# Autodesk Inventor assembly: LegAssembly
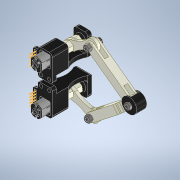
[picture p0: Inventor's stored thumbnail of the model, 180x180]
Saved by Autodesk Inventor 2022 (Build 260153000, 153)
## iProperties
Created: 2021-12-08
Part Number: LegAssembly
Document SubType Name: Assembly
Designer: JK
Author: JK
## Documents named in this file (10)
- C:\Users\JK\Documents\Inventor\N20 Leg Actuator\N20-Leg-Actuator\CADfiles\N20 Leg\LegAssembly.iam
- C:\Users\JK\Documents\Inventor\N20 Leg Actuator\N20-Leg-Actuator\CADfiles\N20Module\N20Module.iam
- C:\Users\JK\Documents\Inventor\N20 Leg Actuator\N20-Leg-Actuator\CADfiles\N20 Leg\ShortLink.ipt
- C:\Users\JK\Documents\Inventor\N20 Leg Actuator\N20-Leg-Actuator\CADfiles\N20 Leg\683zz.ipt
- C:\Users\JK\Documents\Inventor\N20 Leg Actuator\N20-Leg-Actuator\CADfiles\N20 Leg\LinkB.ipt
- C:\Users\JK\Documents\Inventor\N20 Leg Actuator\N20-Leg-Actuator\CADfiles\N20 Leg\LinkA.ipt
- C:\Users\JK\Documents\Inventor\N20 Leg Actuator\N20-Leg-Actuator\CADfiles\N20Module\N20Module_MIR.iam
- C:\Users\JK\Documents\Inventor\N20 Leg Actuator\N20-Leg-Actuator\CADfiles\N20 Leg\M3x12SocketBolt.ipt
- C:\Users\JK\Documents\Inventor\N20 Leg Actuator\N20-Leg-Actuator\CADfiles\N20 Leg\M3 Locknut.ipt
- C:\Users\JK\Documents\Inventor\N20 Leg Actuator\N20-Leg-Actuator\CADfiles\N20 Leg\Rubberfoot.ipt
## Components (16 placed, 9 different names)
1. N20Module:1 [sub-assembly] — Coincidencia:1, Coincidencia:2, Coincidencia:3, Nivelación:6, Nivelación:7, Coincidencia:19
2. ShortLink:1 — Coincidencia:1, Coincidencia:2, Coincidencia:3, Coincidencia:4, Nivelación:1
3. 683zz:1 — Coincidencia:4, Nivelación:1, Coincidencia:10, Coincidencia:11
4. 683zz:2 — Coincidencia:9, Coincidencia:13, Coincidencia:14, Nivelación:5
5. ShortLink:2 — Coincidencia:9, Nivelación:5, Coincidencia:20, Coincidencia:22
6. LinkB:1 — Coincidencia:10, Coincidencia:11, Coincidencia:12, Nivelación:4, Coincidencia:24, Coincidencia:28, Coincidencia:34
7. 683zz:3 — Coincidencia:12, Nivelación:4, Coincidencia:15, Coincidencia:21
8. LinkA:1 — Coincidencia:13, Coincidencia:14, Coincidencia:15, Coincidencia:21, Coincidencia:23, Coincidencia:25, Coincidencia:26, Coincidencia:27, Coincidencia:32, Coincidencia:33, Coincidencia:35, Coincidencia:36, Ángulo:1
9. N20Module_MIR:1 [sub-assembly] — Nivelación:6, Nivelación:7, Coincidencia:19, Coincidencia:20, Coincidencia:22
10. M3x12SocketBolt:1 — Coincidencia:24, Coincidencia:28, Coincidencia:29
11. M3x12SocketBolt:2 — Coincidencia:23, Coincidencia:27, Coincidencia:30
12. M3x12SocketBolt:3 — Coincidencia:25, Coincidencia:26, Coincidencia:31
13. M3 Locknut:1 — Coincidencia:29, Coincidencia:34
14. M3 Locknut:2 — Coincidencia:30, Coincidencia:33
15. M3 Locknut:3 — Coincidencia:31, Coincidencia:32
16. Rubberfoot:1 — Coincidencia:35, Coincidencia:36, Ángulo:1
## Relationships (35: Mate 29, Flush 5, Angle 1)
- Coincidencia:1 [Mate] (0.1 mm): N20Module:1 ↔ ShortLink:1
- Coincidencia:2 [Mate] (0.1 mm): N20Module:1 ↔ ShortLink:1
- Coincidencia:3 [Mate] (0.1 mm): N20Module:1 ↔ ShortLink:1
- Coincidencia:4 [Mate]: ShortLink:1 ↔ 683zz:1
- Nivelación:1 [Flush]: ShortLink:1 ↔ 683zz:1
- Coincidencia:9 [Mate]: 683zz:2 ↔ ShortLink:2
- Coincidencia:10 [Mate]: 683zz:1 ↔ LinkB:1
- Coincidencia:11 [Mate] (0.1 mm): 683zz:1 ↔ LinkB:1
- Coincidencia:12 [Mate]: LinkB:1 ↔ 683zz:3
- Nivelación:4 [Flush]: LinkB:1 ↔ 683zz:3
- Coincidencia:13 [Mate]: 683zz:2 ↔ LinkA:1
- Coincidencia:14 [Mate] (0.1 mm): 683zz:2 ↔ LinkA:1
- Nivelación:5 [Flush]: 683zz:2 ↔ ShortLink:2
- Coincidencia:15 [Mate]: 683zz:3 ↔ LinkA:1
- Nivelación:6 [Flush]: N20Module:1 ↔ N20Module_MIR:1
- Nivelación:7 [Flush]: N20Module:1 ↔ N20Module_MIR:1
- Coincidencia:19 [Mate] (3.7 mm): N20Module:1 ↔ N20Module_MIR:1
- Coincidencia:20 [Mate] (0.1 mm): ShortLink:2 ↔ N20Module_MIR:1
- Coincidencia:21 [Mate]: 683zz:3 ↔ LinkA:1
- Coincidencia:22 [Mate] (0.1 mm): ShortLink:2 ↔ N20Module_MIR:1
- Coincidencia:23 [Mate]: LinkA:1 ↔ M3x12SocketBolt:2
- Coincidencia:24 [Mate]: LinkB:1 ↔ M3x12SocketBolt:1
- Coincidencia:25 [Mate]: LinkA:1 ↔ M3x12SocketBolt:3
- Coincidencia:26 [Mate]: LinkA:1 ↔ M3x12SocketBolt:3
- Coincidencia:27 [Mate]: LinkA:1 ↔ M3x12SocketBolt:2
- Coincidencia:28 [Mate]: LinkB:1 ↔ M3x12SocketBolt:1
- Coincidencia:29 [Mate]: M3x12SocketBolt:1 ↔ M3 Locknut:1
- Coincidencia:30 [Mate]: M3x12SocketBolt:2 ↔ M3 Locknut:2
- Coincidencia:31 [Mate]: M3x12SocketBolt:3 ↔ M3 Locknut:3
- Coincidencia:32 [Mate]: LinkA:1 ↔ M3 Locknut:3
- Coincidencia:33 [Mate]: LinkA:1 ↔ M3 Locknut:2
- Coincidencia:34 [Mate]: LinkB:1 ↔ M3 Locknut:1
- Coincidencia:35 [Mate]: LinkA:1 ↔ Rubberfoot:1
- Coincidencia:36 [Mate]: LinkA:1 ↔ Rubberfoot:1
- Ángulo:1 [Angle] (120 deg): LinkA:1 ↔ Rubberfoot:1
